# Autodesk Inventor assembly: Gripper V1.2
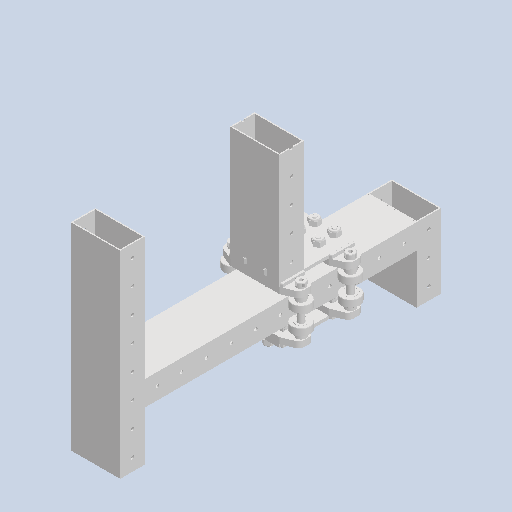
[picture p0: Inventor's stored thumbnail of the model, 512x512]
Saved by Autodesk Inventor 2023 (Build 270158000, 158)
## iProperties
Created: 2023-01-18
Part Number: Gripper V1.2
Document SubType Name: Assembly
Designer: Gabriel - T3 CAD
Author: Gabriel - T3 CAD
## Documents named in this file (8)
- C:\Users\Gabriel - T3 CAD\Documents\GitHub\t3-CAD\T3-CAD\Current Season CAD\Swerve-DriveTrain-V2.1 (LongBot)\Gripper V1.2.iam
- C:\Users\Gabriel - T3 CAD\Documents\GitHub\t3-CAD\T3-CAD\Current Season CAD\Swerve-DriveTrain-V2.1 (LongBot)\Gripper Slider Connecting Plate.ipt
- C:\Users\Gabriel - T3 CAD\Documents\GitHub\t3-CAD\T3-CAD\Stock\ThriftyBot-Elevator\OLD\New folder\Sliding Elevator Block Assembly _1_.iam
- C:\Users\Gabriel - T3 CAD\Documents\GitHub\t3-CAD\T3-CAD\Stock\ThriftyBot-Elevator\OLD\New folder\Sliding Elevator Block Assembly _2_.iam
- C:\Users\Gabriel - T3 CAD\Documents\GitHub\t3-CAD\T3-CAD\Current Season CAD\Swerve-DriveTrain-V2.1 (LongBot)\VersaFrame (Gripper-BaseBar).ipt
- C:\Users\Gabriel - T3 CAD\Documents\GitHub\t3-CAD\T3-CAD\Current Season CAD\Swerve-DriveTrain-V2.1 (LongBot)\VersaFrame (Gripper-StationaryLong).ipt
- C:\Users\Gabriel - T3 CAD\Documents\GitHub\t3-CAD\T3-CAD\Current Season CAD\Swerve-DriveTrain-V2.1 (LongBot)\VersaFrame (Gripper-MovingLong).ipt
- C:\Users\Gabriel - T3 CAD\Documents\GitHub\t3-CAD\T3-CAD\Current Season CAD\Swerve-DriveTrain-V2.1 (LongBot)\VersaFrame (Griper Track Spacer Bar).ipt
## Components (10 placed, 7 different names)
1. Gripper Slider Connecting Plate:1 — Mate:1, Mate:2, Mate:3, Mate:4, Mate:5, Mate:6, Mate:17, Mate:18
2. Sliding Elevator Block Assembly _1_:1 [sub-assembly] — Mate:4, Mate:5, Mate:6, Tangent:2, Tangent:7
3. Sliding Elevator Block Assembly _1_:2 [sub-assembly] — Mate:1, Mate:2, Mate:3, Mate:13, Mate:14, Tangent:1, Tangent:5
4. Sliding Elevator Block Assembly _2_:1 [sub-assembly] — Mate:7, Mate:9, Mate:10, Mate:13, Mate:14, Tangent:4, Tangent:6
5. Sliding Elevator Block Assembly _2_:2 [sub-assembly] — Mate:8, Mate:11, Mate:12, Tangent:3
6. Gripper Slider Connecting Plate:2 — Mate:7, Mate:8, Mate:9, Mate:10, Mate:11, Mate:12
7. VersaFrame (Gripper-BaseBar):1 — Tangent:1, Tangent:2, Tangent:3, Tangent:4, Tangent:5, Tangent:6, Tangent:7, Mate:19, Flush:1, Mate:20, Mate:21
8. VersaFrame (Gripper-StationaryLong):1 — Mate:19, Flush:1
9. VersaFrame (Gripper-MovingLong):1 — Mate:17, Mate:18
10. VersaFrame (Griper Track Spacer Bar):1 — Mate:20, Mate:21
## Relationships (27: Mate 19, Tangent 7, Flush 1)
- Mate:1: Gripper Slider Connecting Plate:1 ↔ Sliding Elevator Block Assembly _1_:2
- Mate:2: Gripper Slider Connecting Plate:1 ↔ Sliding Elevator Block Assembly _1_:2
- Mate:3: Gripper Slider Connecting Plate:1 ↔ Sliding Elevator Block Assembly _1_:2
- Mate:4: Gripper Slider Connecting Plate:1 ↔ Sliding Elevator Block Assembly _1_:1
- Mate:5: Gripper Slider Connecting Plate:1 ↔ Sliding Elevator Block Assembly _1_:1
- Mate:6: Gripper Slider Connecting Plate:1 ↔ Sliding Elevator Block Assembly _1_:1
- Mate:7: Sliding Elevator Block Assembly _2_:1 ↔ Gripper Slider Connecting Plate:2
- Mate:8: Sliding Elevator Block Assembly _2_:2 ↔ Gripper Slider Connecting Plate:2
- Mate:9: Sliding Elevator Block Assembly _2_:1 ↔ Gripper Slider Connecting Plate:2
- Mate:10: Sliding Elevator Block Assembly _2_:1 ↔ Gripper Slider Connecting Plate:2
- Mate:11: Sliding Elevator Block Assembly _2_:2 ↔ Gripper Slider Connecting Plate:2
- Mate:12: Sliding Elevator Block Assembly _2_:2 ↔ Gripper Slider Connecting Plate:2
- Mate:13: Sliding Elevator Block Assembly _1_:2 ↔ Sliding Elevator Block Assembly _2_:1
- Mate:14: Sliding Elevator Block Assembly _1_:2 ↔ Sliding Elevator Block Assembly _2_:1
- Tangent:1: Sliding Elevator Block Assembly _1_:2 ↔ VersaFrame (Gripper-BaseBar):1
- Tangent:2: Sliding Elevator Block Assembly _1_:1 ↔ VersaFrame (Gripper-BaseBar):1
- Tangent:3: Sliding Elevator Block Assembly _2_:2 ↔ VersaFrame (Gripper-BaseBar):1
- Tangent:4: Sliding Elevator Block Assembly _2_:1 ↔ VersaFrame (Gripper-BaseBar):1
- Tangent:5: Sliding Elevator Block Assembly _1_:2 ↔ VersaFrame (Gripper-BaseBar):1
- Tangent:6: Sliding Elevator Block Assembly _2_:1 ↔ VersaFrame (Gripper-BaseBar):1
- Tangent:7: Sliding Elevator Block Assembly _1_:1 ↔ VersaFrame (Gripper-BaseBar):1
- Mate:17: Gripper Slider Connecting Plate:1 ↔ VersaFrame (Gripper-MovingLong):1
- Mate:18: Gripper Slider Connecting Plate:1 ↔ VersaFrame (Gripper-MovingLong):1
- Mate:19: VersaFrame (Gripper-BaseBar):1 ↔ VersaFrame (Gripper-StationaryLong):1
- Flush:1 (50.8 mm): VersaFrame (Gripper-BaseBar):1 ↔ VersaFrame (Gripper-StationaryLong):1
- Mate:20: VersaFrame (Gripper-BaseBar):1 ↔ VersaFrame (Griper Track Spacer Bar):1
- Mate:21: VersaFrame (Gripper-BaseBar):1 ↔ VersaFrame (Griper Track Spacer Bar):1
